# Autodesk Inventor assembly: carriage
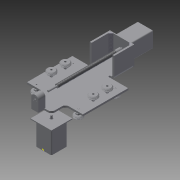
[picture p0: Inventor's stored thumbnail of the model, 180x180]
Saved by Autodesk Inventor 2013 (Build 170138000, 138)
## iProperties
Created: 2012-12-03
Part Number: carriage
Document SubType Name: Weldment
Designer: Istvan
Weld Material: Aluminum 6061, Welded
Mass: 772.809 g
Surface Area: 2087.48 cm^2
Volume: 764.052 cm^3
Density: 1.01146 g/cm^3
Author: Istvan
## Documents named in this file (10)
- C:\Users\istvan.burbank\Documents\GitHub\Crown-Fire\CAD\Carriage\carriage.iam
- C:\Users\istvan.burbank\Documents\GitHub\Crown-Fire\CAD\Carriage\backplate.ipt
- C:\Users\istvan.burbank\Documents\GitHub\Crown-Fire\CAD\Hardware\Bearings\DualVee-size2.ipt
- C:\Users\istvan.burbank\Documents\GitHub\Crown-Fire\CAD\Electronics\Motors\G723-280-4.ipt
- C:\Users\istvan.burbank\Documents\GitHub\Crown-Fire\CAD\Carriage\zMotorMount.ipt
- C:\Users\istvan.burbank\Documents\GitHub\Crown-Fire\CAD\Carriage\acmeScrew.ipt
- C:\Users\istvan.burbank\Documents\GitHub\Crown-Fire\CAD\Hardware\motorCoupling.ipt
- C:\Users\istvan.burbank\Documents\GitHub\Crown-Fire\CAD\Carriage\acmeBearingBlock.ipt
- C:\Users\istvan.burbank\Documents\GitHub\Crown-Fire\CAD\Hardware\Bearings\bearing1-4in.ipt
- C:\Users\istvan.burbank\Documents\GitHub\Crown-Fire\CAD\Carriage\motorMount.ipt
## Components (18 placed, 9 different names)
1. backplate:1 — Mate:5, Flush:4, Flush:5, Angle:1, Mate:13, Mate:18, Mate:19, Mate:20, Mate:21, Mate:22, Mate:23, Mate:24, Mate:25, Flush:7, Flush:8, Flush:9, Mate:26
2. DualVee-size2:1 — Mate:18
3. DualVee-size2:2 — Mate:19
4. DualVee-size2:3 — Mate:21
5. DualVee-size2:4 — Mate:20
6. G723-280-4:1 — Mate:6, Mate:7, Mate:8, Mate:10, Flush:6, Angle:1
7. zMotorMount:1 — Mate:5, Flush:4, Flush:5, Mate:6, Mate:7
8. acmeScrew:1 — Mate:9, Mate:10, Flush:6, Mate:11, Mate:12, Mate:16, Mate:17, Mate:29
9. motorCoupling:1 — Mate:8, Mate:9, Mate:11, Mate:29
10. acmeBearingBlock:1 — Mate:12, Mate:13, Mate:14, Mate:15
11. bearing1-4in:1 — Mate:14, Mate:17
12. bearing1-4in:2 — Mate:15, Mate:16
13. DualVee-size2:5 — Mate:24
14. DualVee-size2:6 — Mate:23
15. DualVee-size2:7 — Mate:25
16. DualVee-size2:8 — Mate:22
17. G723-280-4:2 — Mate:27, Mate:28
18. motorMount:1 — Flush:7, Flush:8, Flush:9, Mate:26, Mate:27, Mate:28
## Relationships (32: Mate 25, Flush 6, Angle 1)
- Mate:5: backplate:1 ↔ zMotorMount:1
- Flush:4: backplate:1 ↔ zMotorMount:1
- Flush:5: backplate:1 ↔ zMotorMount:1
- Mate:6: G723-280-4:1 ↔ zMotorMount:1
- Mate:7 (5.08 mm): G723-280-4:1 ↔ zMotorMount:1
- Mate:8: G723-280-4:1 ↔ motorCoupling:1
- Mate:9: acmeScrew:1 ↔ motorCoupling:1
- Mate:10: G723-280-4:1 ↔ acmeScrew:1
- Flush:6: G723-280-4:1 ↔ acmeScrew:1
- Mate:11: acmeScrew:1 ↔ motorCoupling:1
- Angle:1 (0 deg): backplate:1 ↔ G723-280-4:1
- Mate:12: acmeScrew:1 ↔ acmeBearingBlock:1
- Mate:13: backplate:1 ↔ acmeBearingBlock:1
- Mate:14: acmeBearingBlock:1 ↔ bearing1-4in:1
- Mate:15: acmeBearingBlock:1 ↔ bearing1-4in:2
- Mate:16: acmeScrew:1 ↔ bearing1-4in:2
- Mate:17: acmeScrew:1 ↔ bearing1-4in:1
- Mate:18: backplate:1 ↔ DualVee-size2:1
- Mate:19: backplate:1 ↔ DualVee-size2:2
- Mate:20: backplate:1 ↔ DualVee-size2:4
- Mate:21: backplate:1 ↔ DualVee-size2:3
- Mate:22: backplate:1 ↔ DualVee-size2:8
- Mate:23: backplate:1 ↔ DualVee-size2:6
- Mate:24: backplate:1 ↔ DualVee-size2:5
- Mate:25: backplate:1 ↔ DualVee-size2:7
- Flush:7: backplate:1 ↔ motorMount:1
- Flush:8: backplate:1 ↔ motorMount:1
- Flush:9: backplate:1 ↔ motorMount:1
- Mate:26 (50.8 mm): backplate:1 ↔ motorMount:1
- Mate:27 (6.35 mm): G723-280-4:2 ↔ motorMount:1
- Mate:28: G723-280-4:2 ↔ motorMount:1
- Mate:29: acmeScrew:1 ↔ motorCoupling:1
